# Autodesk Inventor assembly: VP-Input-BAG
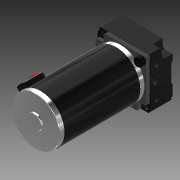
[picture p0: Inventor's stored thumbnail of the model, 180x180]
Saved by Autodesk Inventor 2022 (Build 260153000, 153)
## iProperties
Created: 2018-08-19
Part Number: VP-Input-BAG
Document SubType Name: Assembly
Mass: 418.235 g
Surface Area: 296.022 cm^2
Volume: 114.386 cm^3
Density: 3.65636 g/cm^3
## Documents named in this file (10)
- E:\Middleton Robotics\Collaborative Robots\Collaborative Part Library\General Gearboxes\Planetaries\Versaplanetary\V2 Stages\V2 Input Stage\VP BAG Input.iam
- E:\Middleton Robotics\Collaborative Robots\Collaborative Part Library\General Gearboxes\Planetaries\Versaplanetary\V2 Stages\V2 Input Housing.ipt
- E:\Middleton Robotics\Collaborative Robots\Collaborative Part Library\General Gearboxes\Planetaries\Versaplanetary\Motor Mounting Plates\VP BAG Mounting Plate.ipt
- E:\Middleton Robotics\Collaborative Robots\Collaborative Part Library\General Gearboxes\Planetaries\Versaplanetary\Screws\M4 x 10mm Screw.ipt
- E:\Middleton Robotics\Collaborative Robots\Collaborative Part Library\Motors\FRC\BAG Motor.ipt
- E:\Middleton Robotics\Collaborative Robots\Collaborative Part Library\General Gearboxes\Planetaries\Versaplanetary\Input Coupler\4mm Coupler Sleeve.ipt
- E:\Middleton Robotics\Collaborative Robots\Collaborative Part Library\General Gearboxes\Planetaries\Versaplanetary\Input Coupler\VP Input Coupler.ipt
- E:\Middleton Robotics\Collaborative Robots\Collaborative Part Library\General Gearboxes\Planetaries\Versaplanetary\Input Coupler\Coupler Set Screw.ipt
- E:\Middleton Robotics\Collaborative Robots\Collaborative Part Library\General Gearboxes\Planetaries\Versaplanetary\Screws\8-32 x 0.50in Screw.ipt
- E:\Middleton Robotics\Collaborative Robots\Collaborative Part Library\General Gearboxes\Planetaries\Versaplanetary\V2 Stages\V2 Input Stage.iam
## Components (10 placed, 8 different names)
1. V2 Input Housing:1 — Mate:3, Mate:4, Flush:2, Mate:13, Flush:5, Mate:14, Mate:15
2. VP BAG Mounting Plate:1 — Mate:3, Mate:4, Flush:2, Insert:3, Insert:4, Insert:9, Insert:10, Mate:19
3. M4 x 10mm Screw:1 — Insert:3
4. M4 x 10mm Screw:2 — Insert:4
5. BAG Motor:1 — Insert:9, Insert:10, Insert:13
6. 4mm Coupler Sleeve:1 — Insert:13, Angle:2
7. VP Input Coupler:1 — Mate:12, Tangent:1, Mate:13, Flush:5, Angle:2
8. Coupler Set Screw:1 — Mate:12, Tangent:1
9. 8-32 x 0.50in Screw:1 — Mate:14, Mate:19, Flush:6
10. 8-32 x 0.50in Screw:2 — Mate:15, Flush:6
## Relationships (17: Mate 7, Insert 5, Flush 3, Tangent 1, Angle 1)
- Mate:3: V2 Input Housing:1 ↔ VP BAG Mounting Plate:1
- Mate:4: V2 Input Housing:1 ↔ VP BAG Mounting Plate:1
- Flush:2: V2 Input Housing:1 ↔ VP BAG Mounting Plate:1
- Insert:3: VP BAG Mounting Plate:1 ↔ M4 x 10mm Screw:1
- Insert:4: VP BAG Mounting Plate:1 ↔ M4 x 10mm Screw:2
- Insert:9: VP BAG Mounting Plate:1 ↔ BAG Motor:1
- Insert:10: VP BAG Mounting Plate:1 ↔ BAG Motor:1
- Insert:13: BAG Motor:1 ↔ 4mm Coupler Sleeve:1
- Mate:12: VP Input Coupler:1 ↔ Coupler Set Screw:1
- Tangent:1: VP Input Coupler:1 ↔ Coupler Set Screw:1
- Mate:13: V2 Input Housing:1 ↔ VP Input Coupler:1
- Flush:5 (2.4 mm): V2 Input Housing:1 ↔ VP Input Coupler:1
- Angle:2 (0 deg): 4mm Coupler Sleeve:1 ↔ VP Input Coupler:1
- Mate:14: V2 Input Housing:1 ↔ 8-32 x 0.50in Screw:1
- Mate:15: V2 Input Housing:1 ↔ 8-32 x 0.50in Screw:2
- Mate:19: VP BAG Mounting Plate:1 ↔ 8-32 x 0.50in Screw:1
- Flush:6: 8-32 x 0.50in Screw:1 ↔ 8-32 x 0.50in Screw:2
